# Autodesk Inventor assembly: Stadio10
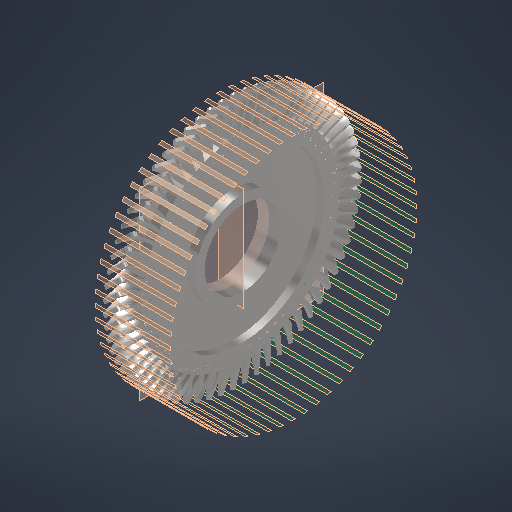
[picture p0: Inventor's stored thumbnail of the model, 512x512]
Saved by Autodesk Inventor 2026.2 (Build 302298010, 298A)
## iProperties
Created: 2026-04-25
Part Number: Stadio10
Document SubType Name: Assembly
Designer: Yan
Author: Yan
## Documents named in this file (3)
- C:\Users\Yan\Desktop\Turbina\Stadio10.iam
- C:\Users\Yan\Desktop\Turbina\DiscoPaleStadio10-DimensioniAprossimate.ipt
- C:\Users\Yan\Desktop\Turbina\PalaStadio10.ipt
## Components (65 placed, 2 different names)
1. DiscoPaleStadio10-DimensioniAprossimate:1 — Mate:1, Mate:2, Mate:3, Mate:4, Mate:5, Mate:6, Mate:7, Mate:8, Mate:9, Mate:10, Mate:11, Mate:12, Mate:13, Mate:14, Mate:15, Mate:16, Mate:17, Mate:18, Mate:19, Mate:20, Mate:21, Mate:22, Mate:23, Mate:24, Mate:25, Mate:26, Mate:27, Mate:28, Mate:29, Mate:30, Mate:31, Mate:32, Mate:33, Mate:34, Mate:35, Mate:36, Mate:37, Mate:38, Mate:39, Mate:40, Mate:41, Mate:42, Mate:43, Mate:44, Mate:45, Mate:46, Mate:47, Mate:48, Mate:49, Mate:50, Mate:51, Mate:52, Mate:53, Mate:54, Mate:55, Mate:56, Mate:57, Mate:58, Mate:59, Mate:60, Mate:61, Mate:62, Mate:63, Mate:64, Mate:65, Mate:66, Mate:67, Mate:68, Mate:69, Mate:70, Mate:71, Mate:72, Mate:73, Mate:74, Mate:75, Mate:76, Mate:77, Mate:78, Mate:79, Mate:80, Mate:81, Mate:82, Mate:83, Mate:84, Mate:85, Mate:86, Mate:87, Mate:88, Mate:89, Mate:90, Mate:91, Mate:92, Mate:93, Mate:94, Mate:95, Mate:96, Mate:97, Mate:98, Mate:99, Mate:100, Mate:101, Mate:102, Mate:103, Mate:104, Mate:105, Mate:106, Mate:107, Mate:108, Mate:109, Mate:110, Mate:111, Mate:112, Mate:113, Mate:114, Flush:1, Flush:2, Flush:3, Flush:4, Flush:5, Flush:6, Flush:7, Flush:8, Flush:9, Flush:10, Flush:11, Flush:12, Flush:13, Flush:14, Flush:15, Flush:16, Flush:17, Flush:18, Flush:19, Flush:20, Flush:21, Flush:22, Flush:23, Flush:24, Flush:25, Flush:26, Flush:27, Flush:28, Flush:29, Flush:30, Flush:31, Flush:32, Flush:33, Flush:34, Flush:35, Flush:36, Flush:37, Flush:38, Flush:39, Flush:40, Flush:41, Flush:42, Flush:43, Flush:44, Flush:45, Flush:46, Flush:47, Flush:48, Flush:49, Flush:50, Flush:51, Flush:52, Flush:53, Flush:54, Flush:55, Flush:56, Flush:57, Flush:58, Flush:59, Flush:60, Flush:61, Flush:62, Flush:63, Mate:115, Mate:116, Mate:117, Mate:118, Mate:119, Mate:120, Mate:121, Mate:122, Mate:123, Mate:124, Mate:125, Mate:126, Mate:127, Flush:64
2. PalaStadio10:1 — Mate:1, Mate:60, Flush:50
3. PalaStadio10:2 — Mate:2, Mate:59, Flush:49
4. PalaStadio10:3 — Mate:3, Mate:58, Flush:48
5. PalaStadio10:4 — Mate:4, Mate:57, Flush:47
6. PalaStadio10:5 — Mate:5, Mate:56, Flush:46
7. PalaStadio10:6 — Mate:6, Mate:55, Flush:45
8. PalaStadio10:7 — Mate:7, Mate:54, Flush:44
9. PalaStadio10:8 — Mate:8, Mate:53, Flush:43
10. PalaStadio10:9 — Mate:9, Mate:52, Flush:42
11. PalaStadio10:10 — Mate:10, Mate:51, Flush:41
12. PalaStadio10:11 — Mate:98, Mate:101, Flush:52
13. PalaStadio10:12 — Mate:19, Mate:42, Flush:32
14. PalaStadio10:13 — Mate:18, Mate:43, Flush:33
15. PalaStadio10:14 — Mate:17, Mate:44, Flush:34
16. PalaStadio10:15 — Mate:16, Mate:45, Flush:35
17. PalaStadio10:16 — Mate:15, Mate:46, Flush:36
18. PalaStadio10:17 — Mate:14, Mate:47, Flush:37
19. PalaStadio10:18 — Mate:13, Mate:48, Flush:38
20. PalaStadio10:19 — Mate:12, Mate:49, Flush:39
21. PalaStadio10:20 — Mate:11, Mate:50, Flush:40
22. PalaStadio10:21 — Mate:91, Mate:108, Flush:59
23. PalaStadio10:22 — Mate:20, Mate:61, Flush:31
24. PalaStadio10:23 — Mate:21, Mate:41, Flush:30
25. PalaStadio10:24 — Mate:22, Mate:40, Flush:29
26. PalaStadio10:25 — Mate:23, Mate:39, Flush:28
27. PalaStadio10:26 — Mate:24, Mate:38, Flush:27
28. PalaStadio10:27 — Mate:25, Mate:37, Flush:26
29. PalaStadio10:28 — Mate:26, Mate:36, Flush:25
30. PalaStadio10:29 — Mate:27, Mate:35, Flush:24
31. PalaStadio10:30 — Mate:28, Mate:34, Flush:23
32. PalaStadio10:31 — Mate:89, Mate:110, Flush:61
33. PalaStadio10:32 — Mate:99, Mate:100, Flush:51
34. PalaStadio10:33 — Mate:87, Mate:112, Flush:63
35. PalaStadio10:34 — Mate:88, Mate:111, Flush:62
36. PalaStadio10:35 — Mate:71, Mate:72, Flush:15
37. PalaStadio10:36 — Mate:65, Mate:69, Flush:18
38. PalaStadio10:37 — Mate:63, Mate:64, Flush:19
39. PalaStadio10:38 — Mate:31, Mate:32, Flush:20
40. PalaStadio10:39 — Mate:30, Mate:33, Flush:21
41. PalaStadio10:40 — Mate:29, Mate:62, Flush:22
42. PalaStadio10:41 — Mate:90, Mate:109, Flush:60
43. PalaStadio10:42 — Mate:86, Mate:113, Flush:1
44. PalaStadio10:43 — Mate:85, Mate:114, Flush:2
45. PalaStadio10:44 — Mate:84, Flush:3
46. PalaStadio10:45 — Mate:83, Flush:4, Mate:125
47. PalaStadio10:46 — Mate:82, Flush:5, Mate:124
48. PalaStadio10:47 — Mate:73, Flush:14, Mate:115
49. PalaStadio10:49 — Mate:67, Mate:70, Flush:16
50. PalaStadio10:50 — Mate:66, Mate:68, Flush:17
51. PalaStadio10:51 — Mate:93, Mate:106, Flush:57
52. PalaStadio10:52 — Mate:92, Mate:107, Flush:58
53. PalaStadio10:53 — Mate:81, Flush:6, Mate:123
54. PalaStadio10:54 — Mate:80, Flush:7, Mate:122
55. PalaStadio10:55 — Mate:79, Flush:8, Mate:121
56. PalaStadio10:56 — Mate:78, Flush:9, Mate:120
57. PalaStadio10:57 — Mate:77, Flush:10, Mate:119
58. PalaStadio10:58 — Mate:76, Flush:11, Mate:118
59. PalaStadio10:59 — Mate:75, Flush:12, Mate:117
60. PalaStadio10:60 — Mate:74, Flush:13, Mate:116
61. PalaStadio10:61 — Mate:94, Mate:105, Flush:56
62. PalaStadio10:62 — Mate:95, Mate:104, Flush:55
63. PalaStadio10:63 — Mate:96, Mate:103, Flush:54
64. PalaStadio10:64 — Mate:97, Mate:102, Flush:53
65. PalaStadio10:65 — Mate:126, Mate:127, Flush:64
## Relationships (191: Mate 127, Flush 64)
- Mate:1: DiscoPaleStadio10-DimensioniAprossimate:1 ↔ PalaStadio10:1
- Mate:2: DiscoPaleStadio10-DimensioniAprossimate:1 ↔ PalaStadio10:2
- Mate:3: DiscoPaleStadio10-DimensioniAprossimate:1 ↔ PalaStadio10:3
- Mate:4: DiscoPaleStadio10-DimensioniAprossimate:1 ↔ PalaStadio10:4
- Mate:5: DiscoPaleStadio10-DimensioniAprossimate:1 ↔ PalaStadio10:5
- Mate:6: DiscoPaleStadio10-DimensioniAprossimate:1 ↔ PalaStadio10:6
- Mate:7: DiscoPaleStadio10-DimensioniAprossimate:1 ↔ PalaStadio10:7
- Mate:8: DiscoPaleStadio10-DimensioniAprossimate:1 ↔ PalaStadio10:8
- Mate:9: DiscoPaleStadio10-DimensioniAprossimate:1 ↔ PalaStadio10:9
- Mate:10: DiscoPaleStadio10-DimensioniAprossimate:1 ↔ PalaStadio10:10
- Mate:11: DiscoPaleStadio10-DimensioniAprossimate:1 ↔ PalaStadio10:20
- Mate:12: DiscoPaleStadio10-DimensioniAprossimate:1 ↔ PalaStadio10:19
- Mate:13: DiscoPaleStadio10-DimensioniAprossimate:1 ↔ PalaStadio10:18
- Mate:14: DiscoPaleStadio10-DimensioniAprossimate:1 ↔ PalaStadio10:17
- Mate:15: DiscoPaleStadio10-DimensioniAprossimate:1 ↔ PalaStadio10:16
- Mate:16: DiscoPaleStadio10-DimensioniAprossimate:1 ↔ PalaStadio10:15
- Mate:17: DiscoPaleStadio10-DimensioniAprossimate:1 ↔ PalaStadio10:14
- Mate:18: DiscoPaleStadio10-DimensioniAprossimate:1 ↔ PalaStadio10:13
- Mate:19: DiscoPaleStadio10-DimensioniAprossimate:1 ↔ PalaStadio10:12
- Mate:20: DiscoPaleStadio10-DimensioniAprossimate:1 ↔ PalaStadio10:22
- Mate:21: DiscoPaleStadio10-DimensioniAprossimate:1 ↔ PalaStadio10:23
- Mate:22: DiscoPaleStadio10-DimensioniAprossimate:1 ↔ PalaStadio10:24
- Mate:23: DiscoPaleStadio10-DimensioniAprossimate:1 ↔ PalaStadio10:25
- Mate:24: DiscoPaleStadio10-DimensioniAprossimate:1 ↔ PalaStadio10:26
- Mate:25: DiscoPaleStadio10-DimensioniAprossimate:1 ↔ PalaStadio10:27
- Mate:26: DiscoPaleStadio10-DimensioniAprossimate:1 ↔ PalaStadio10:28
- Mate:27: DiscoPaleStadio10-DimensioniAprossimate:1 ↔ PalaStadio10:29
- Mate:28: DiscoPaleStadio10-DimensioniAprossimate:1 ↔ PalaStadio10:30
- Mate:29: DiscoPaleStadio10-DimensioniAprossimate:1 ↔ PalaStadio10:40
- Mate:30: DiscoPaleStadio10-DimensioniAprossimate:1 ↔ PalaStadio10:39
- Mate:31: DiscoPaleStadio10-DimensioniAprossimate:1 ↔ PalaStadio10:38
- Mate:32: DiscoPaleStadio10-DimensioniAprossimate:1 ↔ PalaStadio10:38
- Mate:33: DiscoPaleStadio10-DimensioniAprossimate:1 ↔ PalaStadio10:39
- Mate:34: DiscoPaleStadio10-DimensioniAprossimate:1 ↔ PalaStadio10:30
- Mate:35: DiscoPaleStadio10-DimensioniAprossimate:1 ↔ PalaStadio10:29
- Mate:36: DiscoPaleStadio10-DimensioniAprossimate:1 ↔ PalaStadio10:28
- Mate:37: DiscoPaleStadio10-DimensioniAprossimate:1 ↔ PalaStadio10:27
- Mate:38: DiscoPaleStadio10-DimensioniAprossimate:1 ↔ PalaStadio10:26
- Mate:39: DiscoPaleStadio10-DimensioniAprossimate:1 ↔ PalaStadio10:25
- Mate:40: DiscoPaleStadio10-DimensioniAprossimate:1 ↔ PalaStadio10:24
- Mate:41: DiscoPaleStadio10-DimensioniAprossimate:1 ↔ PalaStadio10:23
- Mate:42: DiscoPaleStadio10-DimensioniAprossimate:1 ↔ PalaStadio10:12
- Mate:43: DiscoPaleStadio10-DimensioniAprossimate:1 ↔ PalaStadio10:13
- Mate:44: DiscoPaleStadio10-DimensioniAprossimate:1 ↔ PalaStadio10:14
- Mate:45: DiscoPaleStadio10-DimensioniAprossimate:1 ↔ PalaStadio10:15
- Mate:46: DiscoPaleStadio10-DimensioniAprossimate:1 ↔ PalaStadio10:16
- Mate:47: DiscoPaleStadio10-DimensioniAprossimate:1 ↔ PalaStadio10:17
- Mate:48: DiscoPaleStadio10-DimensioniAprossimate:1 ↔ PalaStadio10:18
- Mate:49: DiscoPaleStadio10-DimensioniAprossimate:1 ↔ PalaStadio10:19
- Mate:50: DiscoPaleStadio10-DimensioniAprossimate:1 ↔ PalaStadio10:20
- Mate:51: DiscoPaleStadio10-DimensioniAprossimate:1 ↔ PalaStadio10:10
- Mate:52: DiscoPaleStadio10-DimensioniAprossimate:1 ↔ PalaStadio10:9
- Mate:53: DiscoPaleStadio10-DimensioniAprossimate:1 ↔ PalaStadio10:8
- Mate:54: DiscoPaleStadio10-DimensioniAprossimate:1 ↔ PalaStadio10:7
- Mate:55: DiscoPaleStadio10-DimensioniAprossimate:1 ↔ PalaStadio10:6
- Mate:56: DiscoPaleStadio10-DimensioniAprossimate:1 ↔ PalaStadio10:5
- Mate:57: DiscoPaleStadio10-DimensioniAprossimate:1 ↔ PalaStadio10:4
- Mate:58: DiscoPaleStadio10-DimensioniAprossimate:1 ↔ PalaStadio10:3
- Mate:59: DiscoPaleStadio10-DimensioniAprossimate:1 ↔ PalaStadio10:2
- Mate:60: DiscoPaleStadio10-DimensioniAprossimate:1 ↔ PalaStadio10:1
- Mate:61: DiscoPaleStadio10-DimensioniAprossimate:1 ↔ PalaStadio10:22
- Mate:62: DiscoPaleStadio10-DimensioniAprossimate:1 ↔ PalaStadio10:40
- Mate:63: DiscoPaleStadio10-DimensioniAprossimate:1 ↔ PalaStadio10:37
- Mate:64: DiscoPaleStadio10-DimensioniAprossimate:1 ↔ PalaStadio10:37
- Mate:65: DiscoPaleStadio10-DimensioniAprossimate:1 ↔ PalaStadio10:36
- Mate:66: DiscoPaleStadio10-DimensioniAprossimate:1 ↔ PalaStadio10:50
- Mate:67: DiscoPaleStadio10-DimensioniAprossimate:1 ↔ PalaStadio10:49
- Mate:68: DiscoPaleStadio10-DimensioniAprossimate:1 ↔ PalaStadio10:50
- Mate:69: DiscoPaleStadio10-DimensioniAprossimate:1 ↔ PalaStadio10:36
- Mate:70: DiscoPaleStadio10-DimensioniAprossimate:1 ↔ PalaStadio10:49
- Mate:71: DiscoPaleStadio10-DimensioniAprossimate:1 ↔ PalaStadio10:35
- Mate:72: DiscoPaleStadio10-DimensioniAprossimate:1 ↔ PalaStadio10:35
- Mate:73: DiscoPaleStadio10-DimensioniAprossimate:1 ↔ PalaStadio10:47
- Mate:74: DiscoPaleStadio10-DimensioniAprossimate:1 ↔ PalaStadio10:60
- Mate:75: DiscoPaleStadio10-DimensioniAprossimate:1 ↔ PalaStadio10:59
- Mate:76: DiscoPaleStadio10-DimensioniAprossimate:1 ↔ PalaStadio10:58
- Mate:77: DiscoPaleStadio10-DimensioniAprossimate:1 ↔ PalaStadio10:57
- Mate:78: DiscoPaleStadio10-DimensioniAprossimate:1 ↔ PalaStadio10:56
- Mate:79: DiscoPaleStadio10-DimensioniAprossimate:1 ↔ PalaStadio10:55
- Mate:80: DiscoPaleStadio10-DimensioniAprossimate:1 ↔ PalaStadio10:54
- Mate:81: DiscoPaleStadio10-DimensioniAprossimate:1 ↔ PalaStadio10:53
- Mate:82: DiscoPaleStadio10-DimensioniAprossimate:1 ↔ PalaStadio10:46
- Mate:83: DiscoPaleStadio10-DimensioniAprossimate:1 ↔ PalaStadio10:45
- Mate:84: DiscoPaleStadio10-DimensioniAprossimate:1 ↔ PalaStadio10:44
- Mate:85: DiscoPaleStadio10-DimensioniAprossimate:1 ↔ PalaStadio10:43
- Mate:86: DiscoPaleStadio10-DimensioniAprossimate:1 ↔ PalaStadio10:42
- Mate:87: DiscoPaleStadio10-DimensioniAprossimate:1 ↔ PalaStadio10:33
- Mate:88: DiscoPaleStadio10-DimensioniAprossimate:1 ↔ PalaStadio10:34
- Mate:89: DiscoPaleStadio10-DimensioniAprossimate:1 ↔ PalaStadio10:31
- Mate:90: DiscoPaleStadio10-DimensioniAprossimate:1 ↔ PalaStadio10:41
- Mate:91: DiscoPaleStadio10-DimensioniAprossimate:1 ↔ PalaStadio10:21
- Mate:92: DiscoPaleStadio10-DimensioniAprossimate:1 ↔ PalaStadio10:52
- Mate:93: DiscoPaleStadio10-DimensioniAprossimate:1 ↔ PalaStadio10:51
- Mate:94: DiscoPaleStadio10-DimensioniAprossimate:1 ↔ PalaStadio10:61
- Mate:95: DiscoPaleStadio10-DimensioniAprossimate:1 ↔ PalaStadio10:62
- Mate:96: DiscoPaleStadio10-DimensioniAprossimate:1 ↔ PalaStadio10:63
- Mate:97: DiscoPaleStadio10-DimensioniAprossimate:1 ↔ PalaStadio10:64
- Mate:98: DiscoPaleStadio10-DimensioniAprossimate:1 ↔ PalaStadio10:11
- Mate:99: DiscoPaleStadio10-DimensioniAprossimate:1 ↔ PalaStadio10:32
- Mate:100: DiscoPaleStadio10-DimensioniAprossimate:1 ↔ PalaStadio10:32
- Mate:101: DiscoPaleStadio10-DimensioniAprossimate:1 ↔ PalaStadio10:11
- Mate:102: DiscoPaleStadio10-DimensioniAprossimate:1 ↔ PalaStadio10:64
- Mate:103: DiscoPaleStadio10-DimensioniAprossimate:1 ↔ PalaStadio10:63
- Mate:104: DiscoPaleStadio10-DimensioniAprossimate:1 ↔ PalaStadio10:62
- Mate:105: DiscoPaleStadio10-DimensioniAprossimate:1 ↔ PalaStadio10:61
- Mate:106: DiscoPaleStadio10-DimensioniAprossimate:1 ↔ PalaStadio10:51
- Mate:107: DiscoPaleStadio10-DimensioniAprossimate:1 ↔ PalaStadio10:52
- Mate:108: DiscoPaleStadio10-DimensioniAprossimate:1 ↔ PalaStadio10:21
- Mate:109: DiscoPaleStadio10-DimensioniAprossimate:1 ↔ PalaStadio10:41
- Mate:110: DiscoPaleStadio10-DimensioniAprossimate:1 ↔ PalaStadio10:31
- Mate:111: DiscoPaleStadio10-DimensioniAprossimate:1 ↔ PalaStadio10:34
- Mate:112: DiscoPaleStadio10-DimensioniAprossimate:1 ↔ PalaStadio10:33
- Mate:113: DiscoPaleStadio10-DimensioniAprossimate:1 ↔ PalaStadio10:42
- Mate:114: DiscoPaleStadio10-DimensioniAprossimate:1 ↔ PalaStadio10:43
- Flush:1: DiscoPaleStadio10-DimensioniAprossimate:1 ↔ PalaStadio10:42
- Flush:2: DiscoPaleStadio10-DimensioniAprossimate:1 ↔ PalaStadio10:43
- Flush:3: DiscoPaleStadio10-DimensioniAprossimate:1 ↔ PalaStadio10:44
- Flush:4: DiscoPaleStadio10-DimensioniAprossimate:1 ↔ PalaStadio10:45
- Flush:5: DiscoPaleStadio10-DimensioniAprossimate:1 ↔ PalaStadio10:46
- Flush:6: DiscoPaleStadio10-DimensioniAprossimate:1 ↔ PalaStadio10:53
- Flush:7: DiscoPaleStadio10-DimensioniAprossimate:1 ↔ PalaStadio10:54
- Flush:8: DiscoPaleStadio10-DimensioniAprossimate:1 ↔ PalaStadio10:55
- Flush:9: DiscoPaleStadio10-DimensioniAprossimate:1 ↔ PalaStadio10:56
- Flush:10: DiscoPaleStadio10-DimensioniAprossimate:1 ↔ PalaStadio10:57
- Flush:11: DiscoPaleStadio10-DimensioniAprossimate:1 ↔ PalaStadio10:58
- Flush:12: DiscoPaleStadio10-DimensioniAprossimate:1 ↔ PalaStadio10:59
- Flush:13: DiscoPaleStadio10-DimensioniAprossimate:1 ↔ PalaStadio10:60
- Flush:14: DiscoPaleStadio10-DimensioniAprossimate:1 ↔ PalaStadio10:47
- Flush:15: DiscoPaleStadio10-DimensioniAprossimate:1 ↔ PalaStadio10:35
- Flush:16: DiscoPaleStadio10-DimensioniAprossimate:1 ↔ PalaStadio10:49
- Flush:17: DiscoPaleStadio10-DimensioniAprossimate:1 ↔ PalaStadio10:50
- Flush:18: DiscoPaleStadio10-DimensioniAprossimate:1 ↔ PalaStadio10:36
- Flush:19: DiscoPaleStadio10-DimensioniAprossimate:1 ↔ PalaStadio10:37
- Flush:20: DiscoPaleStadio10-DimensioniAprossimate:1 ↔ PalaStadio10:38
- Flush:21: DiscoPaleStadio10-DimensioniAprossimate:1 ↔ PalaStadio10:39
- Flush:22: DiscoPaleStadio10-DimensioniAprossimate:1 ↔ PalaStadio10:40
- Flush:23: DiscoPaleStadio10-DimensioniAprossimate:1 ↔ PalaStadio10:30
- Flush:24: DiscoPaleStadio10-DimensioniAprossimate:1 ↔ PalaStadio10:29
- Flush:25: DiscoPaleStadio10-DimensioniAprossimate:1 ↔ PalaStadio10:28
- Flush:26: DiscoPaleStadio10-DimensioniAprossimate:1 ↔ PalaStadio10:27
- Flush:27: DiscoPaleStadio10-DimensioniAprossimate:1 ↔ PalaStadio10:26
- Flush:28: DiscoPaleStadio10-DimensioniAprossimate:1 ↔ PalaStadio10:25
- Flush:29: DiscoPaleStadio10-DimensioniAprossimate:1 ↔ PalaStadio10:24
- Flush:30: DiscoPaleStadio10-DimensioniAprossimate:1 ↔ PalaStadio10:23
- Flush:31: DiscoPaleStadio10-DimensioniAprossimate:1 ↔ PalaStadio10:22
- Flush:32: DiscoPaleStadio10-DimensioniAprossimate:1 ↔ PalaStadio10:12
- Flush:33: DiscoPaleStadio10-DimensioniAprossimate:1 ↔ PalaStadio10:13
- Flush:34: DiscoPaleStadio10-DimensioniAprossimate:1 ↔ PalaStadio10:14
- Flush:35: DiscoPaleStadio10-DimensioniAprossimate:1 ↔ PalaStadio10:15
- Flush:36: DiscoPaleStadio10-DimensioniAprossimate:1 ↔ PalaStadio10:16
- Flush:37: DiscoPaleStadio10-DimensioniAprossimate:1 ↔ PalaStadio10:17
- Flush:38: DiscoPaleStadio10-DimensioniAprossimate:1 ↔ PalaStadio10:18
- Flush:39: DiscoPaleStadio10-DimensioniAprossimate:1 ↔ PalaStadio10:19
- Flush:40: DiscoPaleStadio10-DimensioniAprossimate:1 ↔ PalaStadio10:20
- Flush:41: DiscoPaleStadio10-DimensioniAprossimate:1 ↔ PalaStadio10:10
- Flush:42: DiscoPaleStadio10-DimensioniAprossimate:1 ↔ PalaStadio10:9
- Flush:43: DiscoPaleStadio10-DimensioniAprossimate:1 ↔ PalaStadio10:8
- Flush:44: DiscoPaleStadio10-DimensioniAprossimate:1 ↔ PalaStadio10:7
- Flush:45: DiscoPaleStadio10-DimensioniAprossimate:1 ↔ PalaStadio10:6
- Flush:46: DiscoPaleStadio10-DimensioniAprossimate:1 ↔ PalaStadio10:5
- Flush:47: DiscoPaleStadio10-DimensioniAprossimate:1 ↔ PalaStadio10:4
- Flush:48: DiscoPaleStadio10-DimensioniAprossimate:1 ↔ PalaStadio10:3
- Flush:49: DiscoPaleStadio10-DimensioniAprossimate:1 ↔ PalaStadio10:2
- Flush:50: DiscoPaleStadio10-DimensioniAprossimate:1 ↔ PalaStadio10:1
- Flush:51: DiscoPaleStadio10-DimensioniAprossimate:1 ↔ PalaStadio10:32
- Flush:52: DiscoPaleStadio10-DimensioniAprossimate:1 ↔ PalaStadio10:11
- Flush:53: DiscoPaleStadio10-DimensioniAprossimate:1 ↔ PalaStadio10:64
- Flush:54: DiscoPaleStadio10-DimensioniAprossimate:1 ↔ PalaStadio10:63
- Flush:55: DiscoPaleStadio10-DimensioniAprossimate:1 ↔ PalaStadio10:62
- Flush:56: DiscoPaleStadio10-DimensioniAprossimate:1 ↔ PalaStadio10:61
- Flush:57: DiscoPaleStadio10-DimensioniAprossimate:1 ↔ PalaStadio10:51
- Flush:58: DiscoPaleStadio10-DimensioniAprossimate:1 ↔ PalaStadio10:52
- Flush:59: DiscoPaleStadio10-DimensioniAprossimate:1 ↔ PalaStadio10:21
- Flush:60: DiscoPaleStadio10-DimensioniAprossimate:1 ↔ PalaStadio10:41
- Flush:61: DiscoPaleStadio10-DimensioniAprossimate:1 ↔ PalaStadio10:31
- Flush:62: DiscoPaleStadio10-DimensioniAprossimate:1 ↔ PalaStadio10:34
- Flush:63: DiscoPaleStadio10-DimensioniAprossimate:1 ↔ PalaStadio10:33
- Mate:115: DiscoPaleStadio10-DimensioniAprossimate:1 ↔ PalaStadio10:47
- Mate:116: DiscoPaleStadio10-DimensioniAprossimate:1 ↔ PalaStadio10:60
- Mate:117: DiscoPaleStadio10-DimensioniAprossimate:1 ↔ PalaStadio10:59
- Mate:118: DiscoPaleStadio10-DimensioniAprossimate:1 ↔ PalaStadio10:58
- Mate:119: DiscoPaleStadio10-DimensioniAprossimate:1 ↔ PalaStadio10:57
- Mate:120: DiscoPaleStadio10-DimensioniAprossimate:1 ↔ PalaStadio10:56
- Mate:121: DiscoPaleStadio10-DimensioniAprossimate:1 ↔ PalaStadio10:55
- Mate:122: DiscoPaleStadio10-DimensioniAprossimate:1 ↔ PalaStadio10:54
- Mate:123: DiscoPaleStadio10-DimensioniAprossimate:1 ↔ PalaStadio10:53
- Mate:124: DiscoPaleStadio10-DimensioniAprossimate:1 ↔ PalaStadio10:46
- Mate:125: DiscoPaleStadio10-DimensioniAprossimate:1 ↔ PalaStadio10:45
- Mate:126: DiscoPaleStadio10-DimensioniAprossimate:1 ↔ PalaStadio10:65
- Mate:127: DiscoPaleStadio10-DimensioniAprossimate:1 ↔ PalaStadio10:65
- Flush:64: DiscoPaleStadio10-DimensioniAprossimate:1 ↔ PalaStadio10:65
